# Autodesk Inventor assembly: mew
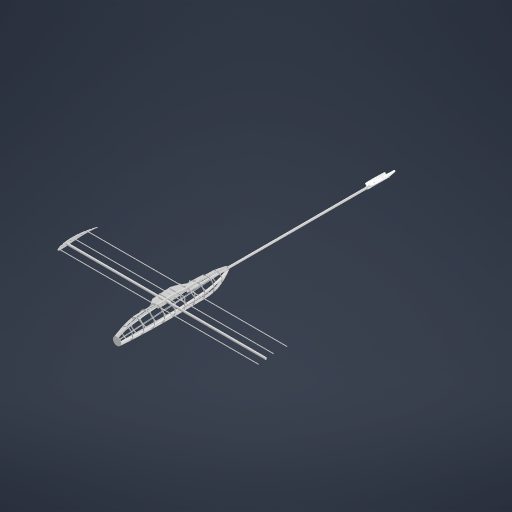
[picture p0: Inventor's stored thumbnail of the model, 512x512]
Saved by Autodesk Inventor 2023.2 (Build 272271000, 271)
## iProperties
Created: 2023-01-02
Part Number: mew
Document SubType Name: Assembly
Designer: Maciej
Author: Maciej
## Documents named in this file (6)
- C:\Users\Maciej\Desktop\samolot\Solaris\main\new model\mew.iam
- C:\Users\Maciej\Desktop\samolot\Solaris\main\new model\kadłub.ipt
- C:\Users\Maciej\Desktop\samolot\Solaris\main\new model\wingspar.ipt
- C:\Users\Maciej\Desktop\samolot\Solaris\main\new model\Tmount.ipt
- C:\Users\Maciej\Desktop\samolot\Solaris\main\new model\small carbon tube.ipt
- C:\Users\Maciej\Desktop\samolot\Solaris\main\new model\Żero montaż.ipt
## Components (8 placed, 5 different names)
1. kadłub:1 — Rigid:1, Rigid:2, Rigid:3, Rigid:4, Rigid:5
2. wingspar:1 — Rigid:2, Mate:6, Flush:1
3. wingspar:2 — Mate:2, Mate:3, Rigid:1
4. Tmount:1 — Mate:2, Mate:3
5. small carbon tube:1 — Rigid:5, Mate:7
6. small carbon tube:2 — Rigid:3, Mate:4
7. small carbon tube:3 — Rigid:4, Mate:5
8. Żero montaż:1 — Mate:4, Mate:5, Mate:6, Mate:7, Flush:1
## Relationships (12: Mate 6, WeldJoint 5, Flush 1)
- Mate:2: wingspar:2 ↔ Tmount:1
- Mate:3: wingspar:2 ↔ Tmount:1
- Rigid:1 [WeldJoint] (-300 mm): kadłub:1 ↔ wingspar:2
- Rigid:2 [WeldJoint] (0.75 mm): kadłub:1 ↔ wingspar:1
- Rigid:3 [WeldJoint] (-0.75 mm): kadłub:1 ↔ small carbon tube:2
- Rigid:4 [WeldJoint] (0.75 mm): kadłub:1 ↔ small carbon tube:3
- Rigid:5 [WeldJoint] (0.75 mm): kadłub:1 ↔ small carbon tube:1
- Mate:4: small carbon tube:2 ↔ Żero montaż:1
- Mate:5: small carbon tube:3 ↔ Żero montaż:1
- Mate:6: wingspar:1 ↔ Żero montaż:1
- Mate:7: small carbon tube:1 ↔ Żero montaż:1
- Flush:1: wingspar:1 ↔ Żero montaż:1
